# Autodesk Inventor assembly: Base
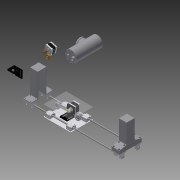
[picture p0: Inventor's stored thumbnail of the model, 180x180]
Saved by Autodesk Inventor 2015 (Build 190159000, 159)
## iProperties
Created: 2015-02-24
Part Number: Base
Document SubType Name: Assembly
Designer: Andrew
Author: Andrew
## Documents named in this file (14)
- C:\Users\pltwe4\Documents\model\Base.iam
- C:\Users\pltwe4\Documents\model\Linear Bearing Platform Small.ipt
- C:\Users\pltwe4\Documents\model\Base Plate.ipt
- C:\Users\pltwe4\Documents\model\NEMA 17 Stepper.ipt
- C:\Users\pltwe4\Documents\model\GT2 Pulley.ipt
- C:\Users\pltwe4\Documents\model\Stepper Motor Mount.ipt
- C:\Users\pltwe4\Documents\model\MainRod.ipt
- C:\Users\pltwe4\Documents\model\Linear Rail Shaft Guide.ipt
- C:\Users\pltwe4\Documents\model\Belt Tensioner Assy.iam
- C:\Users\pltwe4\Documents\model\X-Ray Tube.ipt
- C:\Users\pltwe4\Documents\model\Compression Arm.ipt
- C:\Users\pltwe4\Documents\model\Spur Gear.ipt
- C:\Users\pltwe4\Documents\model\Worm Gear.ipt
- C:\Users\pltwe4\Documents\model\Sheet Metal Arm v2.ipt
## Components (28 placed, 13 different names)
1. Linear Bearing Platform Small:1 — Flush:5, Mate:7, Flush:9, Flush:11, Flush:12
2. Linear Bearing Platform Small:2 — Flush:4, Flush:5, Flush:6, Mate:6, Angle:2, Flush:8, Flush:10
3. Linear Bearing Platform Small:3 — Flush:4, Mate:8, Flush:8
4. Linear Bearing Platform Small:4 — Flush:6, Mate:1, Mate:9, Angle:3, Flush:9, Flush:13
5. Base Plate:1 — Flush:1, Flush:2, Flush:3, Mate:1, Mate:5, Angle:2, Angle:3, Flush:10, Flush:11, Flush:12, Flush:13, Angle:4, Flush:26, Flush:27, Mate:24, Flush:30
6. NEMA 17 Stepper:1 — Mate:4, Flush:7, Angle:1, Mate:14, Mate:15
7. GT2 Pulley:1 — Mate:4, Flush:7, Mate:22
8. Stepper Motor Mount:1 — Angle:1, Mate:5, Angle:4, Mate:14, Mate:15, Flush:30
9. MainRod:1 — Mate:6, Mate:7, Mate:10, Flush:16, Mate:12, Mate:17, Mate:19, Flush:24
10. MainRod:2 — Mate:8, Mate:9, Mate:11, Flush:16, Mate:13, Mate:16, Mate:18, Flush:23
11. Linear Rail Shaft Guide:1 — Mate:10, Flush:14, Flush:15, Mate:20, Flush:24, Mate:31
12. Linear Rail Shaft Guide:2 — Mate:11, Flush:14, Flush:15
13. Linear Rail Shaft Guide:3 — Mate:12, Mate:21, Mate:25
14. Linear Rail Shaft Guide:4 — Mate:13, Flush:23, Flush:29
15. Linear Rail Shaft Guide:5 — Mate:17, Mate:21, Symmetry:1, Flush:28
16. Linear Rail Shaft Guide:6 — Mate:16, Symmetry:1
17. Linear Rail Shaft Guide:7 — Mate:19, Mate:20, Mate:29, Mate:30
18. Linear Rail Shaft Guide:8 — Mate:18
19. Belt Tensioner Assy:1 [sub-assembly] — Flush:25, Mate:23
20. Belt Tensioner Assy:2 [sub-assembly] — Flush:25
21. Base Plate:2 — Flush:26, Flush:27, Mate:24
22. X-Ray Tube:1
23. Compression Arm:1 — Flush:28, Flush:29, Mate:25
24. Spur Gear:1
25. Stepper Motor Mount:2
26. Worm Gear:1 — Mate:27, Mate:28
27. NEMA 17 Stepper:2 — Mate:27, Mate:28
28. Sheet Metal Arm v2:1 — Mate:29, Mate:30, Mate:31
## Relationships (63: Flush 30, Mate 28, Angle 4, Symmetry 1)
- Flush:1: Base Plate:1
- Flush:2: Base Plate:1
- Flush:3: Base Plate:1
- Flush:4: Linear Bearing Platform Small:2 ↔ Linear Bearing Platform Small:3
- Flush:5: Linear Bearing Platform Small:1 ↔ Linear Bearing Platform Small:2
- Flush:6: Linear Bearing Platform Small:2 ↔ Linear Bearing Platform Small:4
- Mate:1: Linear Bearing Platform Small:4 ↔ Base Plate:1
- Mate:4: NEMA 17 Stepper:1 ↔ GT2 Pulley:1
- Flush:7: NEMA 17 Stepper:1 ↔ GT2 Pulley:1
- Angle:1 (0 deg): NEMA 17 Stepper:1 ↔ Stepper Motor Mount:1
- Mate:5 (10 mm): Base Plate:1 ↔ Stepper Motor Mount:1
- Mate:6: Linear Bearing Platform Small:2 ↔ MainRod:1
- Mate:7: Linear Bearing Platform Small:1 ↔ MainRod:1
- Mate:8: Linear Bearing Platform Small:3 ↔ MainRod:2
- Mate:9: Linear Bearing Platform Small:4 ↔ MainRod:2
- Mate:10: MainRod:1 ↔ Linear Rail Shaft Guide:1
- Mate:11: MainRod:2 ↔ Linear Rail Shaft Guide:2
- Angle:2 (0 deg): Linear Bearing Platform Small:2 ↔ Base Plate:1
- Angle:3 (0 deg): Linear Bearing Platform Small:4 ↔ Base Plate:1
- Flush:8: Linear Bearing Platform Small:2 ↔ Linear Bearing Platform Small:3
- Flush:9: Linear Bearing Platform Small:1 ↔ Linear Bearing Platform Small:4
- Flush:10 (5 mm): Linear Bearing Platform Small:2 ↔ Base Plate:1
- Flush:11 (5 mm): Linear Bearing Platform Small:1 ↔ Base Plate:1
- Flush:12 (5 mm): Linear Bearing Platform Small:1 ↔ Base Plate:1
- Flush:13 (5 mm): Linear Bearing Platform Small:4 ↔ Base Plate:1
- Flush:14: Linear Rail Shaft Guide:1 ↔ Linear Rail Shaft Guide:2
- Flush:15: Linear Rail Shaft Guide:1 ↔ Linear Rail Shaft Guide:2
- Flush:16: MainRod:1 ↔ MainRod:2
- Angle:4 (180 deg): Base Plate:1 ↔ Stepper Motor Mount:1
- [Flush]: Linear Rail Shaft Guide:3 ↔ Linear Rail Shaft Guide:4
- [Flush]: Linear Rail Shaft Guide:3 ↔ Linear Rail Shaft Guide:4
- Mate:12: MainRod:1 ↔ Linear Rail Shaft Guide:3
- Mate:13: MainRod:2 ↔ Linear Rail Shaft Guide:4
- Mate:14: NEMA 17 Stepper:1 ↔ Stepper Motor Mount:1
- Mate:15: NEMA 17 Stepper:1 ↔ Stepper Motor Mount:1
- [Flush]: Linear Rail Shaft Guide:5 ↔ Linear Rail Shaft Guide:6
- [Flush]: Linear Rail Shaft Guide:5 ↔ Linear Rail Shaft Guide:6
- Mate:16: MainRod:2 ↔ Linear Rail Shaft Guide:6
- Mate:17: MainRod:1 ↔ Linear Rail Shaft Guide:5
- [Flush]: Linear Rail Shaft Guide:7 ↔ Linear Rail Shaft Guide:8
- [Flush]: Linear Rail Shaft Guide:7 ↔ Linear Rail Shaft Guide:8
- Mate:18: MainRod:2 ↔ Linear Rail Shaft Guide:8
- Mate:19: MainRod:1 ↔ Linear Rail Shaft Guide:7
- Mate:20 (20 mm): Linear Rail Shaft Guide:1 ↔ Linear Rail Shaft Guide:7
- Mate:21 (20 mm): Linear Rail Shaft Guide:3 ↔ Linear Rail Shaft Guide:5
- Flush:23 (5 mm): MainRod:2 ↔ Linear Rail Shaft Guide:4
- Flush:24 (5 mm): MainRod:1 ↔ Linear Rail Shaft Guide:1
- Symmetry:1: Linear Rail Shaft Guide:5 ↔ Linear Rail Shaft Guide:6
- Mate:22: GT2 Pulley:1
- Flush:25: Belt Tensioner Assy:1 ↔ Belt Tensioner Assy:2
- Mate:23: Belt Tensioner Assy:1
- Flush:26: Base Plate:1 ↔ Base Plate:2
- Flush:27: Base Plate:1 ↔ Base Plate:2
- Mate:24 (65 mm): Base Plate:1 ↔ Base Plate:2
- Flush:28: Linear Rail Shaft Guide:5 ↔ Compression Arm:1
- Flush:29: Linear Rail Shaft Guide:4 ↔ Compression Arm:1
- Mate:25: Linear Rail Shaft Guide:3 ↔ Compression Arm:1
- Mate:27: Worm Gear:1 ↔ NEMA 17 Stepper:2
- Mate:28 (3 mm): Worm Gear:1 ↔ NEMA 17 Stepper:2
- Mate:29: Linear Rail Shaft Guide:7 ↔ Sheet Metal Arm v2:1
- Mate:30: Linear Rail Shaft Guide:7 ↔ Sheet Metal Arm v2:1
- Mate:31: Linear Rail Shaft Guide:1 ↔ Sheet Metal Arm v2:1
- Flush:30: Base Plate:1 ↔ Stepper Motor Mount:1
## Named parameters: d31_d27 = 0 mm, d32_d28 = 0 mm, d37_d31_d27 = 0 mm, d38_d32_d28 = 0 mm, d41_d27 = 0 mm, d42_d28 = 0 mm
